# Autodesk Inventor assembly: 車軸受け
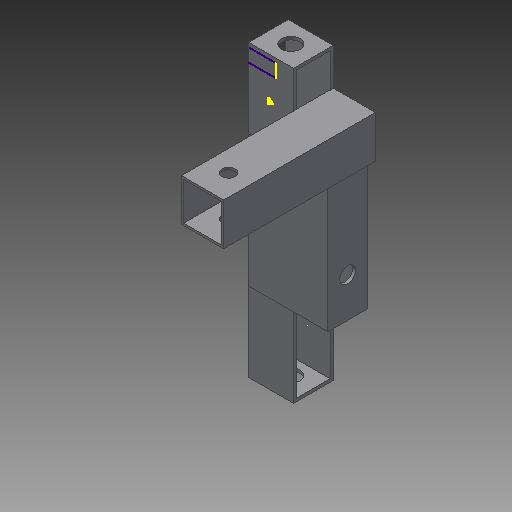
[picture p0: Inventor's stored thumbnail of the model, 512x512]
Saved by Autodesk Inventor 2018 (Build 220112000, 112)
## iProperties
Created: 2017-09-15
Part Number: 車軸受け
Material: 一般
Document SubType Name: Assembly
Designer: mura5
Author: mura5
## Documents named in this file (4)
- C:\Users\mura5\Documents\RBBR\CAD\サスペンション\車軸受け(前,右).iam
- C:\Users\mura5\Documents\RBBR\CAD\サスペンション\車軸受け1.ipt
- C:\Users\mura5\Documents\RBBR\CAD\サスペンション\車軸受け2.ipt
- C:\Users\mura5\Documents\RBBR\CAD\サスペンション\車軸受け4.ipt
## Components (4 placed, 3 different names)
1. 車軸受け1:1 — リジッド:1, リジッド:2
2. 車軸受け2:1 — リジッド:1, リジッド:3
3. 車軸受け2:2 — リジッド:2
4. 車軸受け4:1 — リジッド:3
## Relationships (3: WeldJoint 3)
- リジッド:1 [WeldJoint]: 車軸受け1:1 ↔ 車軸受け2:1
- リジッド:2 [WeldJoint]: 車軸受け1:1 ↔ 車軸受け2:2
- リジッド:3 [WeldJoint]: 車軸受け2:1 ↔ 車軸受け4:1
